# Autodesk Inventor assembly: grabber shoulder hinge
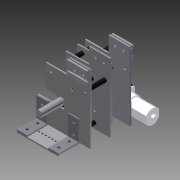
[picture p0: Inventor's stored thumbnail of the model, 180x180]
Saved by Autodesk Inventor 2011 SP1 (Build 150282100, 282)
## iProperties
Created: 2011-01-12
Part Number: grabber shoulder hinge
Document SubType Name: Assembly
Designer: Christopher
Author: Christopher
## Documents named in this file (14)
- C:\Users\Christopher\Documents\Christopher\FIRST\Inventor files\2011\linlifterarm\grabber shoulder hinge.iam
- C:\Users\Christopher\Documents\Christopher\FIRST\Inventor files\2011\Kit of Parts\motors\Motors_Denso_262100-3030.ipt
- C:\Users\Christopher\Documents\Christopher\FIRST\Inventor files\2011\Kit of Parts\motors\Motors_Pelham Plastics_Denso-6.ipt
- C:\Users\Christopher\Documents\Christopher\FIRST\Inventor files\2011\linlifterarm\AS5-8-5-001.ipt
- C:\Users\Christopher\Documents\Christopher\FIRST\Inventor files\2011\linlifterarm\AD-hoc .625 spacer.ipt
- C:\Users\Christopher\Documents\Christopher\FIRST\Inventor files\2011\linlifterarm\AS5-8-4-001.ipt
- C:\Users\Christopher\Documents\Christopher\FIRST\Inventor files\2011\linlifterarm\Ad-Hoc 5!8 keyed axle.ipt
- C:\Users\Christopher\Documents\Christopher\FIRST\Inventor files\2011\linlifterarm\Ad-hoc 3!16 axle key.ipt
- C:\Users\Christopher\Documents\Christopher\FIRST\Inventor files\2011\linlifterarm\AD-hoc 1.125 spacer.ipt
- C:\Users\Christopher\Documents\Christopher\FIRST\Inventor files\2011\linlifterarm\AS5-8-5-002.ipt
- C:\Users\Christopher\Documents\Christopher\FIRST\Inventor files\2011\linlifterarm\AD-hoc 1.75 spacer.ipt
- C:\Users\Christopher\Documents\Christopher\FIRST\Inventor files\2011\Kit of Parts\plastic bearings\NK04-40 CARRIAGE.ipt
- C:\Users\Christopher\Documents\Christopher\FIRST\Inventor files\2011\linlifterarm\Ad-hoc 2 by 1 angle bracket.ipt
- C:\Users\Christopher\Documents\Christopher\FIRST\Inventor files\2011\linlifterarm\AS2-8-4-001.ipt
## Components (24 placed, 13 different names)
1. Motors_Denso_262100-3030:1 — Insert:1, Insert:2, Insert:3, Insert:11
2. Motors_Pelham Plastics_Denso-6:1 — Insert:1, Mate:3, Mate:4
3. AS5-8-5-001:1 — Insert:2, Insert:3, Insert:4, Insert:6, Insert:7, Mate:6, Flush:3, Flush:4
4. AD-hoc .625 spacer:1 — Insert:4, Insert:10
5. AD-hoc .625 spacer:2 — Insert:7, Insert:8
6. AD-hoc .625 spacer:3 — Insert:6, Insert:9
7. AS5-8-4-001:1 — Insert:8, Insert:9, Insert:10, Insert:12, Insert:13, Insert:14, Insert:15
8. Ad-Hoc 5!8 keyed axle:1 — Insert:11
9. Ad-hoc 3!16 axle key:1 — Mate:3, Mate:4
10. AD-hoc 1.125 spacer:1 — Insert:14
11. AD-hoc 1.125 spacer:2 — Insert:13
12. AD-hoc 1.125 spacer:3 — Insert:15
13. AD-hoc 1.125 spacer:4 — Insert:12
14. AS5-8-5-002:1 — Insert:20, Insert:21, Insert:22, Insert:23
15. AD-hoc 1.75 spacer:1 — Insert:22, Insert:25
16. AD-hoc 1.75 spacer:2 — Insert:21, Insert:26
17. AD-hoc 1.75 spacer:3 — Insert:20, Insert:24
18. AD-hoc 1.75 spacer:4 — Insert:23, Insert:27
19. AS5-8-5-002:2 — Insert:24, Insert:25, Insert:26, Insert:27, Mate:5, Flush:1, Flush:2, Insert:28, Insert:29, Insert:30, Insert:31
20. NK04-40 CARRIAGE:1 — Mate:6, Flush:3, Flush:4
21. NK04-40 CARRIAGE:2 — Mate:5, Flush:1, Flush:2
22. Ad-hoc 2 by 1 angle bracket:1 — Insert:28, Insert:29, Insert:32, Insert:34
23. Ad-hoc 2 by 1 angle bracket:2 — Insert:30, Insert:31, Insert:33, Insert:35
24. AS2-8-4-001:1 — Insert:32, Insert:33, Insert:34, Insert:35
## Relationships (38: Insert 30, Mate 4, Flush 4)
- Insert:1: Motors_Denso_262100-3030:1 ↔ Motors_Pelham Plastics_Denso-6:1
- Insert:2: Motors_Denso_262100-3030:1 ↔ AS5-8-5-001:1
- Insert:3: Motors_Denso_262100-3030:1 ↔ AS5-8-5-001:1
- Insert:4: AS5-8-5-001:1 ↔ AD-hoc .625 spacer:1
- Insert:6: AS5-8-5-001:1 ↔ AD-hoc .625 spacer:3
- Insert:7: AS5-8-5-001:1 ↔ AD-hoc .625 spacer:2
- Insert:8: AD-hoc .625 spacer:2 ↔ AS5-8-4-001:1
- Insert:9: AD-hoc .625 spacer:3 ↔ AS5-8-4-001:1
- Insert:10: AD-hoc .625 spacer:1 ↔ AS5-8-4-001:1
- Mate:3: Motors_Pelham Plastics_Denso-6:1 ↔ Ad-hoc 3!16 axle key:1
- Mate:4: Motors_Pelham Plastics_Denso-6:1 ↔ Ad-hoc 3!16 axle key:1
- Insert:11: Motors_Denso_262100-3030:1 ↔ Ad-Hoc 5!8 keyed axle:1
- Insert:12: AS5-8-4-001:1 ↔ AD-hoc 1.125 spacer:4
- Insert:13: AS5-8-4-001:1 ↔ AD-hoc 1.125 spacer:2
- Insert:14: AS5-8-4-001:1 ↔ AD-hoc 1.125 spacer:1
- Insert:15: AS5-8-4-001:1 ↔ AD-hoc 1.125 spacer:3
- Insert:20: AS5-8-5-002:1 ↔ AD-hoc 1.75 spacer:3
- Insert:21: AS5-8-5-002:1 ↔ AD-hoc 1.75 spacer:2
- Insert:22: AS5-8-5-002:1 ↔ AD-hoc 1.75 spacer:1
- Insert:23: AS5-8-5-002:1 ↔ AD-hoc 1.75 spacer:4
- Insert:24: AD-hoc 1.75 spacer:3 ↔ AS5-8-5-002:2
- Insert:25: AD-hoc 1.75 spacer:1 ↔ AS5-8-5-002:2
- Insert:26: AD-hoc 1.75 spacer:2 ↔ AS5-8-5-002:2
- Insert:27: AD-hoc 1.75 spacer:4 ↔ AS5-8-5-002:2
- Mate:5: AS5-8-5-002:2 ↔ NK04-40 CARRIAGE:2
- Flush:1: AS5-8-5-002:2 ↔ NK04-40 CARRIAGE:2
- Flush:2: AS5-8-5-002:2 ↔ NK04-40 CARRIAGE:2
- Mate:6: AS5-8-5-001:1 ↔ NK04-40 CARRIAGE:1
- Flush:3: AS5-8-5-001:1 ↔ NK04-40 CARRIAGE:1
- Flush:4: AS5-8-5-001:1 ↔ NK04-40 CARRIAGE:1
- Insert:28: AS5-8-5-002:2 ↔ Ad-hoc 2 by 1 angle bracket:1
- Insert:29: AS5-8-5-002:2 ↔ Ad-hoc 2 by 1 angle bracket:1
- Insert:30: AS5-8-5-002:2 ↔ Ad-hoc 2 by 1 angle bracket:2
- Insert:31: AS5-8-5-002:2 ↔ Ad-hoc 2 by 1 angle bracket:2
- Insert:32: Ad-hoc 2 by 1 angle bracket:1 ↔ AS2-8-4-001:1
- Insert:33: Ad-hoc 2 by 1 angle bracket:2 ↔ AS2-8-4-001:1
- Insert:34: Ad-hoc 2 by 1 angle bracket:1 ↔ AS2-8-4-001:1
- Insert:35: Ad-hoc 2 by 1 angle bracket:2 ↔ AS2-8-4-001:1
